# Autodesk Inventor assembly: GE-13019
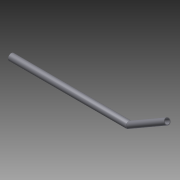
[picture p0: Inventor's stored thumbnail of the model, 180x180]
Saved by Autodesk Inventor 2013 (Build 170138000, 138)
## iProperties
Created: 2013-01-06
Part Number: GE-13019
Document SubType Name: Assembly
Designer: Phillip
_SolveAssemblyDoc: Frame Generator Solve Assembly
_Version: 15.0.0
Author: Phillip
## Documents named in this file (3)
- C:\Users\Moses\Documents\Inventor\2013 Team 3061 Robot\FIRST Arena 2013\Pyramid\GE-13019.iam
- C:\Users\Moses\Documents\Inventor\2013 Team 3061 Robot\FIRST Arena 2013\Pyramid\GE-13019-1Frame.ipt
- C:\Users\Moses\Documents\Inventor\2013 Team 3061 Robot\FIRST Arena 2013\Pyramid\GE-13019\Frame\Frame0001.iam
## Components (2 placed, 2 different names)
1. GE-13019-1Frame:1
2. Frame0001:1 [sub-assembly] — Mate:1, Flush:1
## Relationships (4: Mate 3, Flush 1)
- Mate:1: Frame0001:1
- Flush:1: Frame0001:1
- Mate:2
- Mate:3
